# Autodesk Inventor assembly: _MK-1_Assembly
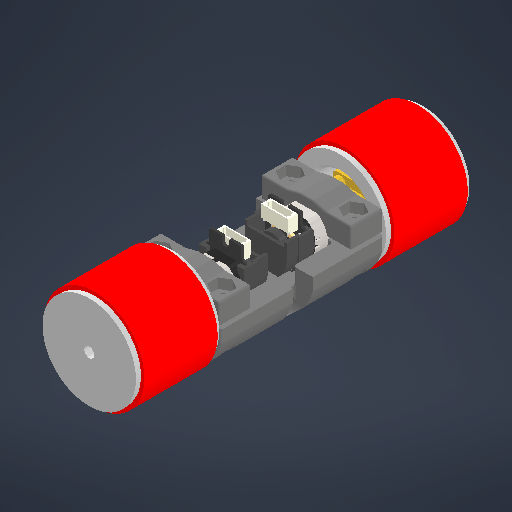
[picture p0: Inventor's stored thumbnail of the model, 512x512]
Saved by Autodesk Inventor 2026.2 (Build 302298010, 298A)
## iProperties
Created: 2026-03-30
Part Number: _MK-1_Assembly
Document SubType Name: Assembly
Designer: zak
Author: zak
## Documents named in this file (6)
- C:\Users\zak\GitHub\NeoSumec-MiniSumo-MECH\_MK-1_\_MK-1_Assembly.iam
- C:\Users\zak\GitHub\NeoSumec-MiniSumo-MECH\_MK-1_\3D_Print\MotorMountBottom.ipt
- C:\Users\zak\GitHub\NeoSumec-MiniSumo-MECH\_MK-1_\3rd-party_comp\Pololu Micro Metal Gearmotor 3D (STEP) Models\With Encoder, Side Connector\mmgm-cb-enc-side-con\mmgm-cb-enc-side-con\mmgm-cb-enc-side-con.ipt
- C:\Users\zak\GitHub\NeoSumec-MiniSumo-MECH\_MK-1_\3D_Print\MotorClamp.ipt
- C:\Users\zak\GitHub\NeoSumec-MiniSumo-MECH\_MK-1_\Metal\Wheel.ipt
- C:\Users\zak\GitHub\NeoSumec-MiniSumo-MECH\_MK-1_\Other technology\silicon bublebum.ipt
## Components (9 placed, 5 different names)
1. MotorMountBottom:1 — Stejný směr:1, Proti sobě:1, Stejný směr:2, Proti sobě:2, Proti sobě:4, Proti sobě:5, Proti sobě:7, Proti sobě:8, Proti sobě:13, Proti sobě:18
2. mmgm-cb-enc-side-con:1 — Stejný směr:2, Proti sobě:2, Proti sobě:3, Proti sobě:9, Proti sobě:10
3. mmgm-cb-enc-side-con:2 — Stejný směr:1, Proti sobě:1, Proti sobě:6, Proti sobě:16, Proti sobě:17
4. MotorClamp:1 — Proti sobě:6, Proti sobě:7, Proti sobě:8
5. MotorClamp:2 — Proti sobě:3, Proti sobě:4, Proti sobě:5
6. Wheel:1 — Proti sobě:14, Proti sobě:15, Proti sobě:16, Proti sobě:17, Proti sobě:18
7. Wheel:2 — Proti sobě:9, Proti sobě:10, Proti sobě:11, Proti sobě:12, Proti sobě:13
8. silicon bublebum:1 — Proti sobě:11, Proti sobě:12
9. silicon bublebum:2 — Proti sobě:14, Proti sobě:15
## Relationships (20: Mate 18, Flush 2)
- Stejný směr:1 [Flush] (-5 mm): MotorMountBottom:1 ↔ mmgm-cb-enc-side-con:2
- Proti sobě:1 [Mate]: MotorMountBottom:1 ↔ mmgm-cb-enc-side-con:2
- Stejný směr:2 [Flush] (-5 mm): MotorMountBottom:1 ↔ mmgm-cb-enc-side-con:1
- Proti sobě:2 [Mate]: MotorMountBottom:1 ↔ mmgm-cb-enc-side-con:1
- Proti sobě:3 [Mate]: mmgm-cb-enc-side-con:1 ↔ MotorClamp:2
- Proti sobě:4 [Mate]: MotorMountBottom:1 ↔ MotorClamp:2
- Proti sobě:5 [Mate]: MotorMountBottom:1 ↔ MotorClamp:2
- Proti sobě:6 [Mate]: mmgm-cb-enc-side-con:2 ↔ MotorClamp:1
- Proti sobě:7 [Mate]: MotorMountBottom:1 ↔ MotorClamp:1
- Proti sobě:8 [Mate]: MotorMountBottom:1 ↔ MotorClamp:1
- Proti sobě:9 [Mate]: mmgm-cb-enc-side-con:1 ↔ Wheel:2
- Proti sobě:10 [Mate] (0.1 mm): mmgm-cb-enc-side-con:1 ↔ Wheel:2
- Proti sobě:11 [Mate]: Wheel:2 ↔ silicon bublebum:1
- Proti sobě:12 [Mate]: Wheel:2 ↔ silicon bublebum:1
- Proti sobě:13 [Mate] (0.5 mm): MotorMountBottom:1 ↔ Wheel:2
- Proti sobě:14 [Mate]: Wheel:1 ↔ silicon bublebum:2
- Proti sobě:15 [Mate]: Wheel:1 ↔ silicon bublebum:2
- Proti sobě:16 [Mate]: mmgm-cb-enc-side-con:2 ↔ Wheel:1
- Proti sobě:17 [Mate] (0.25 mm): mmgm-cb-enc-side-con:2 ↔ Wheel:1
- Proti sobě:18 [Mate] (0.5 mm): MotorMountBottom:1 ↔ Wheel:1
